# Autodesk Inventor assembly: David_Mac_Jones
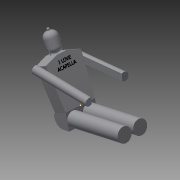
[picture p0: Inventor's stored thumbnail of the model, 180x180]
Saved by Autodesk Inventor 2015 SP1 (Build 190203100, 203)
## iProperties
Created: 2016-02-03
Part Number: David_Mac_Jones
Document SubType Name: Assembly
Designer: guillemd
Author: guillemd
## Documents named in this file (6)
- U:\Mechatronics\Motion Base Rough model\David_Mac_Jones.iam
- U:\Mechatronics\Motion Base Rough model\DMJ_arm.ipt
- U:\Mechatronics\Motion Base Rough model\DMJ_hat.ipt
- U:\Mechatronics\Motion Base Rough model\DMJ_Head.ipt
- U:\Mechatronics\Motion Base Rough model\DMJ_Legs.ipt
- U:\Mechatronics\Motion Base Rough model\DMJ_torso.ipt
## Components (6 placed, 5 different names)
1. DMJ_arm:1 — Mate:7, Angle:2
2. DMJ_arm:2 — Mate:8, Angle:3
3. DMJ_hat:1 — Tangent:1, Angle:1, Mate:3
4. DMJ_Head:1 — Mate:1, Mate:2, Tangent:1, Mate:3
5. DMJ_Legs:1 — Mate:4, Mate:5, Mate:6
6. DMJ_torso:1 — Mate:1, Mate:2, Angle:1, Mate:4, Mate:5, Mate:6, Mate:7, Angle:2, Mate:8, Angle:3
## Relationships (12: Mate 8, Angle 3, Tangent 1)
- Mate:1: DMJ_Head:1 ↔ DMJ_torso:1
- Mate:2: DMJ_Head:1 ↔ DMJ_torso:1
- Tangent:1: DMJ_hat:1 ↔ DMJ_Head:1
- Angle:1 (180 deg): DMJ_hat:1 ↔ DMJ_torso:1
- Mate:3: DMJ_hat:1 ↔ DMJ_Head:1
- Mate:4: DMJ_Legs:1 ↔ DMJ_torso:1
- Mate:5: DMJ_Legs:1 ↔ DMJ_torso:1
- Mate:6: DMJ_Legs:1 ↔ DMJ_torso:1
- Mate:7: DMJ_arm:1 ↔ DMJ_torso:1
- Angle:2 (-30 deg): DMJ_arm:1 ↔ DMJ_torso:1
- Mate:8: DMJ_arm:2 ↔ DMJ_torso:1
- Angle:3 (20 deg): DMJ_arm:2 ↔ DMJ_torso:1
